# Autodesk Inventor assembly: marble_lift
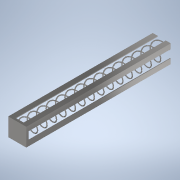
[picture p0: Inventor's stored thumbnail of the model, 180x180]
Saved by Autodesk Inventor 2020 (Build 240168000, 168)
## iProperties
Created: 2021-03-06
Part Number: marble_lift
Document SubType Name: Assembly
Designer: Harry
Author: Harry
## Documents named in this file (3)
- C:\Users\Harry\Documents\hacktheburgh\octocatch\cad\marble_lift.iam
- C:\Users\Harry\Documents\hacktheburgh\octocatch\cad\marble_lift_outer.ipt
- C:\Users\Harry\Documents\hacktheburgh\octocatch\cad\marble_lift_shaft.ipt
## Components (2 placed, 2 different names)
1. marble_lift_outer:1 — Insert:1
2. marble_lift_shaft:1 — Insert:1
## Relationships (1: Insert 1)
- Insert:1: marble_lift_outer:1 ↔ marble_lift_shaft:1
